# Autodesk Inventor assembly: front wheel
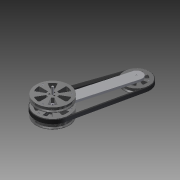
[picture p0: Inventor's stored thumbnail of the model, 180x180]
Saved by Autodesk Inventor 2011 (Build 150239000, 239)
## iProperties
Created: 2010-04-20
Part Number: front wheel
Document SubType Name: Assembly
Designer: lucio
Mass: 1076.54 g
Surface Area: 3619.37 cm^2
Volume: 1073.08 cm^3
Density: 1.00323 g/cm^3
Author: lucio
## Documents named in this file (3)
- C:\Users\lucio\Documents\Inventor\caterpillar\front wheel.iam
- C:\Users\lucio\Documents\Inventor\caterpillar\back wheel.iam
- C:\Users\lucio\Documents\Inventor\caterpillar\font arm.iam
## Components (2 placed, 2 different names)
1. back wheel:1 [sub-assembly] — Mate:1, Mate:2
2. font arm:1 [sub-assembly] — Mate:1, Mate:2
## Relationships (2: Mate 2)
- Mate:1: back wheel:1 ↔ font arm:1
- Mate:2: back wheel:1 ↔ font arm:1
